# Autodesk Inventor assembly: 2018FRCField_rev2
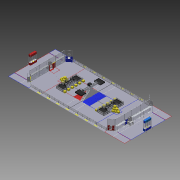
[picture p0: Inventor's stored thumbnail of the model, 180x180]
Saved by Autodesk Inventor 2018 (Build 220112000, 112)
## iProperties
Category: FRC Field 2018
Company: Autodesk Inc.
Created: 2017-12-17
Part Number: 2018FRCField_rev2
Vendor: FIRST Inc.
Document SubType Name: Assembly
Designer: Autodesk Inc.
Author: Autodesk Inc.
Keywords: FRC 2018
## Documents named in this file (32)
- D:\FIRST 2018\FIRST 2018 Inventor\FIRST 2018 Field\FRC Field 2018.iam
- D:\FIRST 2018\FIRST 2018 Inventor\FIRST 2018 Field\Parts\FE-00041-01.ipt
- D:\FIRST 2018\FIRST 2018 Inventor\FIRST 2018 Field\Parts\FE-00041-02.iam
- D:\FIRST 2018\FIRST 2018 Inventor\FIRST 2018 Field\Parts\FE-00041-03.iam
- D:\FIRST 2018\FIRST 2018 Inventor\FIRST 2018 Field\Parts\GE-18112.iam
- D:\FIRST 2018\FIRST 2018 Inventor\FIRST 2018 Field\Parts\GE-18120.iam
- D:\FIRST 2018\FIRST 2018 Inventor\FIRST 2018 Field\Parts\Tape_StartingLine.ipt
- D:\FIRST 2018\FIRST 2018 Inventor\FIRST 2018 Field\Parts\Tape_NullZone.ipt
- D:\FIRST 2018\FIRST 2018 Inventor\FIRST 2018 Field\Parts\GE-18117.ipt
- D:\FIRST 2018\FIRST 2018 Inventor\FIRST 2018 Field\Parts\GE-18118.ipt
- D:\FIRST 2018\FIRST 2018 Inventor\FIRST 2018 Field\Parts\GE-18116.ipt
- D:\FIRST 2018\FIRST 2018 Inventor\FIRST 2018 Field\Parts\GE-18124.ipt
- D:\FIRST 2018\FIRST 2018 Inventor\FIRST 2018 Field\Parts\GE-18126_Blue.iam
- D:\FIRST 2018\FIRST 2018 Inventor\FIRST 2018 Field\Parts\GE-18126_Red.iam
- D:\FIRST 2018\FIRST 2018 Inventor\FIRST 2018 Field\Parts\Tape_AllianceStation_Blue.ipt
- D:\FIRST 2018\FIRST 2018 Inventor\FIRST 2018 Field\Parts\Tape_Portal_Red.ipt
- D:\FIRST 2018\FIRST 2018 Inventor\FIRST 2018 Field\Parts\Tape_ExchangeZone_Red.ipt
- D:\FIRST 2018\FIRST 2018 Inventor\FIRST 2018 Field\Parts\Tape_AutoLine_Blue.ipt
- D:\FIRST 2018\FIRST 2018 Inventor\FIRST 2018 Field\Parts\Tape_PowerCubeZone_Blue.ipt
- D:\FIRST 2018\FIRST 2018 Inventor\FIRST 2018 Field\Parts\Tape_PlatformZone_Blue.ipt
- D:\FIRST 2018\FIRST 2018 Inventor\FIRST 2018 Field\Parts\Tape_PlatformZone_Red.ipt
- D:\FIRST 2018\FIRST 2018 Inventor\FIRST 2018 Field\Parts\Tape_AutoLine_Red.ipt
- D:\FIRST 2018\FIRST 2018 Inventor\FIRST 2018 Field\Parts\Tape_PowerCubeZone_Red.ipt
- D:\FIRST 2018\FIRST 2018 Inventor\FIRST 2018 Field\Parts\Tape_ExchangeZone_Blue.ipt
- D:\FIRST 2018\FIRST 2018 Inventor\FIRST 2018 Field\Parts\Tape_Portal_Blue.ipt
- D:\FIRST 2018\FIRST 2018 Inventor\FIRST 2018 Field\Parts\Tape_AllianceStation_Red.ipt
- D:\FIRST 2018\FIRST 2018 Inventor\FIRST 2018 Field\Parts\GE-18100_Blue.iam
- D:\FIRST 2018\FIRST 2018 Inventor\FIRST 2018 Field\Parts\GE-18100_Red.iam
- D:\FIRST 2018\FIRST 2018 Inventor\FIRST 2018 Field\Parts\GE-18109_Red.iam
- D:\FIRST 2018\FIRST 2018 Inventor\FIRST 2018 Field\Parts\GE-18109_Blue.iam
- D:\FIRST 2018\FIRST 2018 Inventor\FIRST 2018 Field\Parts\GE-18108_Blue.iam
- D:\FIRST 2018\FIRST 2018 Inventor\FIRST 2018 Field\Parts\GE-18108_Red.iam
## Components (79 placed, 79 different names)
1. FE-00041-01_1 — Mate:2, Mate:4, Flush:9, Mate:9, Flush:20, Mate:16, Mate:17, Flush:22, Mate:20, Mate:21
2. FE-00041-01_2 — Mate:1, Mate:3, Flush:6, Flush:7, Flush:8, Mate:6, Flush:10, Flush:11, Mate:10, Flush:12, Flush:13, Flush:14, Mate:11, Flush:15, Mate:12, Flush:17, Flush:18, Mate:13, Flush:19, Mate:14, Mate:15, Flush:21, Mate:18, Mate:19, Flush:23, Mate:23, Mate:24
3. FE-00041-02_3 [sub-assembly]
4. FE-00041-02_4 [sub-assembly]
5. FE-00041-03_5 [sub-assembly]
6. FE-00041-03_6 [sub-assembly]
7. GE-18100_7 [sub-assembly]
8. GE-18100_8 [sub-assembly] — Flush:16
9. GE-18108_9 [sub-assembly]
10. GE-18108_10 [sub-assembly]
11. GE-18109_11 [sub-assembly]
12. GE-18109_12 [sub-assembly]
13. GE-18112_13 [sub-assembly]
14. GE-18112_14 [sub-assembly]
15. GE-18120_15 [sub-assembly]
16. Tape_AllianceStation_16 — Flush:5
17. Tape_Portal_17
18. Tape_Portal_18 — Mate:22
19. Tape_ExchangeZone_19
20. Tape_AutoLine_20
21. Tape_PowerCubeZone_21
22. Tape_StartingLine_22 — Flush:12, Flush:23, Mate:22, Mate:23
23. Tape_PlatformZone_23
24. Tape_NullZone_24 — Flush:19, Mate:14, Mate:15
25. Tape_PlatformZone_25
26. Tape_PlatformZone_26 — Flush:22, Mate:20, Mate:21
27. Tape_PlatformZone_27 — Flush:21, Mate:18, Mate:19
28. Tape_NullZone_28 — Flush:20, Mate:16, Mate:17
29. Tape_AutoLine_29 — Flush:10, Flush:11, Mate:10
30. Tape_PowerCubeZone_30 — Flush:17, Flush:18, Mate:13
31. Tape_ExchangeZone_31 — Flush:15, Flush:16, Mate:12
32. Tape_StartingLine_32 — Flush:13, Flush:14, Mate:11
33. Tape_AllianceStation_33 — Flush:1, Flush:6, Mate:7, Mate:8, Mate:24
34. Tape_Portal_34 — Flush:7, Flush:8, Mate:6, Mate:7
35. Tape_Portal_35 — Flush:9, Mate:8, Mate:9
36. GE-18117_36
37. GE-18118_37
38. GE-18116_38
39. GE-18118_39
40. GE-18117_40
41. GE-18116_41
42. GE-18116_42
43. GE-18116_43
44. GE-18116_44
45. GE-18116_45
46. GE-18124_46
47. GE-18124_47
48. GE-18124_48
49. GE-18124_49
50. GE-18124_50
51. GE-18124_51
52. GE-18124_52
53. GE-18124_53
54. GE-18124_54
55. GE-18124_55
56. GE-18124_56
57. GE-18124_57
58. GE-18124_58
59. GE-18124_59
60. GE-18124_60
61. GE-18124_61
62. GE-18124_62
63. GE-18124_63
64. GE-18124_64
65. GE-18124_65
66. GE-18124_66
67. GE-18124_67
68. GE-18124_68
69. GE-18124_69
70. GE-18124_70
71. GE-18124_71
72. GE-18124_72
73. GE-18124_73
74. GE-18124_74
75. GE-18124_75
76. GE-18124_76
77. GE-18124_77
78. GE-18126_Blue:1 [sub-assembly] — Mate:1, Mate:2, Flush:1
79. GE-18126_Red:1 [sub-assembly] — Mate:3, Flush:5, Mate:4
## Relationships (43: Mate 23, Flush 20)
- Mate:1: FE-00041-01_2 ↔ GE-18126_Blue:1
- Mate:2: FE-00041-01_1 ↔ GE-18126_Blue:1
- Flush:1: Tape_AllianceStation_33 ↔ GE-18126_Blue:1
- Mate:3: FE-00041-01_2 ↔ GE-18126_Red:1
- Flush:5: Tape_AllianceStation_16 ↔ GE-18126_Red:1
- Mate:4: FE-00041-01_1 ↔ GE-18126_Red:1
- Flush:6: FE-00041-01_2 ↔ Tape_AllianceStation_33
- Flush:7: FE-00041-01_2 ↔ Tape_Portal_34
- Flush:8: FE-00041-01_2 ↔ Tape_Portal_34
- Mate:6: FE-00041-01_2 ↔ Tape_Portal_34
- Mate:7: Tape_AllianceStation_33 ↔ Tape_Portal_34
- Flush:9: FE-00041-01_1 ↔ Tape_Portal_35
- Mate:8: Tape_AllianceStation_33 ↔ Tape_Portal_35
- Mate:9: FE-00041-01_1 ↔ Tape_Portal_35
- Flush:10 (-6096 mm): FE-00041-01_2 ↔ Tape_AutoLine_29
- Flush:11 (457.2 mm): FE-00041-01_2 ↔ Tape_AutoLine_29
- Mate:10: FE-00041-01_2 ↔ Tape_AutoLine_29
- Flush:12 (2281.2502 mm): FE-00041-01_2 ↔ Tape_StartingLine_22
- Flush:13 (-2281.2502 mm): FE-00041-01_2 ↔ Tape_StartingLine_32
- Flush:14 (50.8 mm): FE-00041-01_2 ↔ Tape_StartingLine_32
- Mate:11: FE-00041-01_2 ↔ Tape_StartingLine_32
- Flush:15 (-3048 mm): FE-00041-01_2 ↔ Tape_ExchangeZone_31
- Flush:16 (-914.4 mm): GE-18100_8 ↔ Tape_ExchangeZone_31
- Mate:12: FE-00041-01_2 ↔ Tape_ExchangeZone_31
- Flush:17 (4000.5 mm): FE-00041-01_2 ↔ Tape_PowerCubeZone_30
- Flush:18 (5537.2 mm): FE-00041-01_2 ↔ Tape_PowerCubeZone_30
- Mate:13: FE-00041-01_2 ↔ Tape_PowerCubeZone_30
- Flush:19 (10363.2 mm): FE-00041-01_2 ↔ Tape_NullZone_24
- Mate:14 (-2875.7118 mm): FE-00041-01_2 ↔ Tape_NullZone_24
- Mate:15: FE-00041-01_2 ↔ Tape_NullZone_24
- Flush:20 (10363.2 mm): FE-00041-01_1 ↔ Tape_NullZone_28
- Mate:16 (-2875.0006 mm): FE-00041-01_1 ↔ Tape_NullZone_28
- Mate:17: FE-00041-01_1 ↔ Tape_NullZone_28
- Flush:21 (2875.7118 mm): FE-00041-01_2 ↔ Tape_PlatformZone_27
- Mate:18 (-11268.075 mm): FE-00041-01_2 ↔ Tape_PlatformZone_27
- Mate:19: FE-00041-01_2 ↔ Tape_PlatformZone_27
- Flush:22 (-2875.0006 mm): FE-00041-01_1 ↔ Tape_PlatformZone_26
- Mate:20 (-11268.075 mm): FE-00041-01_1 ↔ Tape_PlatformZone_26
- Mate:21: FE-00041-01_1 ↔ Tape_PlatformZone_26
- Flush:23 (2281.2502 mm): FE-00041-01_2 ↔ Tape_StartingLine_22
- Mate:22: Tape_Portal_18 ↔ Tape_StartingLine_22
- Mate:23: FE-00041-01_2 ↔ Tape_StartingLine_22
- Mate:24: FE-00041-01_2 ↔ Tape_AllianceStation_33
